# Autodesk Inventor assembly: Full chassis
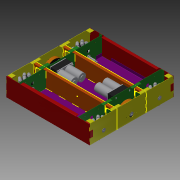
[picture p0: Inventor's stored thumbnail of the model, 180x180]
Saved by Autodesk Inventor 2014 SP1 (Build 180222100, 222)
## iProperties
Created: 2014-01-06
Part Number: Full chassis
Document SubType Name: Weldment
Designer: Alex
Weld Material: Welded Aluminum-6061
Author: Alex
## Documents named in this file (11)
- C:\Users\noah\Documents\Inventor\FRC 2014\Chassis V1\Workspace\V1\Full chassis.iam
- C:\Users\noah\Documents\Inventor\FRC 2014\Chassis V1\Workspace\V1\Front.ipt
- C:\Users\noah\Documents\Inventor\FRC 2014\Chassis V1\Workspace\V1\Outer_Side.ipt
- C:\Users\noah\Documents\Inventor\FRC 2014\Chassis V1\Workspace\V1\InnerSide.ipt
- C:\Users\noah\Documents\Inventor\FRC 2014\Chassis V1\Workspace\V1\Brace.ipt
- C:\Users\noah\Documents\Inventor\FRC 2014\Chassis V1\Workspace\V1\Base.ipt
- C:\Users\noah\Documents\Inventor\FRC 2014\Chassis V1\Workspace\V1\super-shifter-asm-penumatic-hex-long\super-shifter-asm-penumatic-hex-long.iam
- C:\Users\noah\Documents\Inventor\FRC 2014\Chassis V1\Workspace\V1\super-shifter-asm-penumatic-hex-long\fr8zz-hex.ipt
- C:\Users\noah\Documents\Inventor\FRC 2014\Chassis V1\Workspace\V1\super-shifter-asm-penumatic-hex-long\super_d17.ipt
- C:\Users\noah\Documents\Inventor\FRC 2014\Chassis V1\Workspace\V1\Meccanum_VexPro_6in_RH\Meccanum_VexPro_6in_RH.iam
- C:\Users\noah\Documents\Inventor\FRC 2014\Chassis V1\Workspace\V1\6Plaction-asm\6Plaction-asm.iam
## Components (31 placed, 10 different names)
1. Front:1 — Mate:1, Flush:6, Flush:7, Flush:10, Flush:12, Mate:7, Mate:9
2. Outer_Side:1 — Flush:6, Flush:10, Flush:12, Flush:16, Flush:17, Flush:18, Flush:19, Rotational:3, Rotational:7, Rotational:14
3. Outer_Side:2 — Mate:1, Flush:7, Mate:13, Rigid:1, Mate:35, Rotational:1, Rotational:9, Rotational:13
4. InnerSide:2 — Mate:7, Mate:13, Mate:15, Mate:33, Mate:34, Rotational:8, Rotational:10, Mate:36
5. Brace:1 — Flush:16, Flush:17
6. Brace:2 — Mate:9, Flush:18, Flush:19, Mate:12, Mate:27, Mate:28, Mate:29
7. Base:1 — Mate:12, Mate:15
8. Front:2 — Rigid:1
9. InnerSide:3 — Mate:27, Mate:28, Mate:29, Mate:30, Mate:31, Mate:32, Rotational:11, Rotational:12
10. super-shifter-asm-penumatic-hex-long:1 [sub-assembly] — Mate:30, Mate:31, Mate:32, Mate:43
11. super-shifter-asm-penumatic-hex-long:2 [sub-assembly] — Mate:33, Mate:34, Mate:35, Mate:36, Mate:45
12. fr8zz-hex:1 — Rotational:1, Mate:38, Flush:21
13. fr8zz-hex:2 — Rotational:13
14. fr8zz-hex:3 — Rotational:9, Mate:37, Flush:20
15. fr8zz-hex:4 — Rotational:11
16. fr8zz-hex:5 — Rotational:8
17. fr8zz-hex:6 — Rotational:14
18. fr8zz-hex:7 — Rotational:10
19. fr8zz-hex:8 — Rotational:12
20. fr8zz-hex:9 — Rotational:3, Mate:39, Flush:22
21. fr8zz-hex:10 — Rotational:7, Mate:40, Flush:23
22. super_d17:1 — Mate:37, Flush:20, Mate:46
23. super_d17:2 — Mate:39, Flush:22, Mate:41
24. super_d17:3 — Mate:40, Flush:23, Mate:42
25. super_d17:4 — Mate:38, Flush:21, Mate:44
26. Meccanum_VexPro_6in_RH:1 [sub-assembly] — Mate:44
27. Meccanum_VexPro_6in_RH:2 [sub-assembly] — Mate:42
28. Meccanum_VexPro_6in_RH:3 [sub-assembly] — Mate:41
29. Meccanum_VexPro_6in_RH:4 [sub-assembly] — Mate:46
30. 6Plaction-asm:1 [sub-assembly] — Mate:45
31. 6Plaction-asm:2 [sub-assembly] — Mate:43
## Relationships (49: Mate 26, Flush 12, RevoluteJoint 10, WeldJoint 1)
- Mate:1: Front:1 ↔ Outer_Side:2
- Flush:6: Front:1 ↔ Outer_Side:1
- Flush:7: Front:1 ↔ Outer_Side:2
- Flush:10: Front:1 ↔ Outer_Side:1
- Flush:12: Front:1 ↔ Outer_Side:1
- Mate:7: Front:1 ↔ InnerSide:2
- Flush:16: Outer_Side:1 ↔ Brace:1
- Flush:17: Outer_Side:1 ↔ Brace:1
- Mate:9 (-228.6 mm): Front:1 ↔ Brace:2
- Flush:18: Outer_Side:1 ↔ Brace:2
- Flush:19: Outer_Side:1 ↔ Brace:2
- Mate:12: Brace:2 ↔ Base:1
- Mate:13 (-101.6 mm): Outer_Side:2 ↔ InnerSide:2
- Mate:15: InnerSide:2 ↔ Base:1
- Rigid:1 [WeldJoint]: Outer_Side:2 ↔ Front:2
- Mate:27: Brace:2 ↔ InnerSide:3
- Mate:28: Brace:2 ↔ InnerSide:3
- Mate:29: Brace:2 ↔ InnerSide:3
- Mate:30: InnerSide:3 ↔ super-shifter-asm-penumatic-hex-long:1
- Mate:31: InnerSide:3 ↔ super-shifter-asm-penumatic-hex-long:1
- Mate:32: InnerSide:3 ↔ super-shifter-asm-penumatic-hex-long:1
- Mate:33: InnerSide:2 ↔ super-shifter-asm-penumatic-hex-long:2
- Mate:34: InnerSide:2 ↔ super-shifter-asm-penumatic-hex-long:2
- Mate:35: Outer_Side:2 ↔ super-shifter-asm-penumatic-hex-long:2
- Rotational:1 [RevoluteJoint]: Outer_Side:2 ↔ fr8zz-hex:1
- Rotational:3 [RevoluteJoint]: Outer_Side:1 ↔ fr8zz-hex:9
- Rotational:7 [RevoluteJoint]: Outer_Side:1 ↔ fr8zz-hex:10
- Rotational:8 [RevoluteJoint]: InnerSide:2 ↔ fr8zz-hex:5
- Rotational:9 [RevoluteJoint]: Outer_Side:2 ↔ fr8zz-hex:3
- Rotational:10 [RevoluteJoint]: InnerSide:2 ↔ fr8zz-hex:7
- Rotational:11 [RevoluteJoint]: InnerSide:3 ↔ fr8zz-hex:4
- Rotational:12 [RevoluteJoint]: InnerSide:3 ↔ fr8zz-hex:8
- Rotational:13 [RevoluteJoint]: Outer_Side:2 ↔ fr8zz-hex:2
- Rotational:14 [RevoluteJoint]: Outer_Side:1 ↔ fr8zz-hex:6
- Mate:36: InnerSide:2 ↔ super-shifter-asm-penumatic-hex-long:2
- Mate:37: fr8zz-hex:3 ↔ super_d17:1
- Flush:20: fr8zz-hex:3 ↔ super_d17:1
- Mate:38: fr8zz-hex:1 ↔ super_d17:4
- Flush:21: fr8zz-hex:1 ↔ super_d17:4
- Mate:39: fr8zz-hex:9 ↔ super_d17:2
- Flush:22: fr8zz-hex:9 ↔ super_d17:2
- Mate:40: fr8zz-hex:10 ↔ super_d17:3
- Flush:23: fr8zz-hex:10 ↔ super_d17:3
- Mate:41: super_d17:2 ↔ Meccanum_VexPro_6in_RH:3
- Mate:42: super_d17:3 ↔ Meccanum_VexPro_6in_RH:2
- Mate:43: super-shifter-asm-penumatic-hex-long:1 ↔ 6Plaction-asm:2
- Mate:44: super_d17:4 ↔ Meccanum_VexPro_6in_RH:1
- Mate:45: super-shifter-asm-penumatic-hex-long:2 ↔ 6Plaction-asm:1
- Mate:46: super_d17:1 ↔ Meccanum_VexPro_6in_RH:4
